# Autodesk Inventor assembly: Assembly1
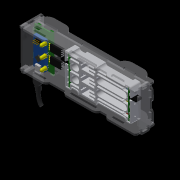
[picture p0: Inventor's stored thumbnail of the model, 180x180]
Saved by Autodesk Inventor 2016 (Build 200138000, 138)
## iProperties
Created: 2015-06-16
Part Number: Assembly1
Document SubType Name: Assembly
Designer: Openlab
Author: Openlab
## Documents named in this file (12)
- D:\Alexey\HS-Spectrophotometer\parts\Paris\Assembly.iam
- D:\Alexey\HS-Spectrophotometer\parts\Paris\Core_bottom.ipt
- D:\Alexey\HS-Spectrophotometer\parts\Paris\LED_board.ipt
- D:\Alexey\HS-Spectrophotometer\parts\Paris\Sensor_board.ipt
- D:\Alexey\HS-Spectrophotometer\parts\Paris\Core_top.ipt
- D:\Alexey\HS-Spectrophotometer\parts\Paris\Box_top.ipt
- D:\Alexey\HS-Spectrophotometer\parts\Paris\Box_bottom.ipt
- D:\Alexey\HS-Spectrophotometer\parts\Paris\Box_left_wall.ipt
- D:\Alexey\HS-Spectrophotometer\parts\Paris\Box_right_wall.ipt
- D:\Alexey\HS-Spectrophotometer\parts\Paris\Microcontroller_board_assumbly.iam
- D:\Alexey\HS-Spectrophotometer\parts\Paris\Box_back_wall.ipt
- D:\Alexey\HS-Spectrophotometer\parts\Paris\Box_front_wall.ipt
## Components (12 placed, 11 different names)
1. Core_bottom:1 — Mate:1, Mate:4, Mate:7, Mate:13, Mate:14, Mate:15, Mate:16, Mate:52, Mate:53, Mate:54, Mate:74
2. LED_board:1 — Mate:4, Mate:13, Mate:14
3. Sensor_board:1 — Mate:7, Mate:15, Mate:16
4. Core_top:1 — Mate:1, Mate:52, Mate:53, Mate:54, Mate:73, Mate:75
5. Box_top:1 — Mate:72, Mate:73, Mate:74, Mate:75, Mate:76, Mate:77, Mate:78, Mate:84, Mate:86, Mate:92
6. Box_bottom:1 — Mate:79, Mate:80, Mate:81
7. Box_left_wall:1 — Mate:83, Mate:84, Mate:85, Mate:91
8. Box_right_wall:1 — Mate:72
9. Microcontroller_board_assumbly:1 [sub-assembly] — Mate:89, Mate:90, Mate:91
10. Box_back_wall:1 — Mate:76, Mate:77, Mate:78, Mate:79, Mate:80, Mate:81, Mate:83, Mate:85, Mate:87, Mate:88
11. Box_front_wall:1 — Mate:92, Mate:93, Mate:94
12. Box_left_wall:2 — Mate:86, Mate:87, Mate:88, Mate:89, Mate:90, Mate:93, Mate:94
## Relationships (32: Mate 32)
- Mate:1: Core_bottom:1 ↔ Core_top:1
- Mate:4: Core_bottom:1 ↔ LED_board:1
- Mate:7: Core_bottom:1 ↔ Sensor_board:1
- Mate:13: Core_bottom:1 ↔ LED_board:1
- Mate:14: Core_bottom:1 ↔ LED_board:1
- Mate:15: Core_bottom:1 ↔ Sensor_board:1
- Mate:16: Core_bottom:1 ↔ Sensor_board:1
- Mate:52: Core_bottom:1 ↔ Core_top:1
- Mate:53: Core_bottom:1 ↔ Core_top:1
- Mate:54: Core_bottom:1 ↔ Core_top:1
- Mate:72: Box_top:1 ↔ Box_right_wall:1
- Mate:73: Core_top:1 ↔ Box_top:1
- Mate:74: Core_bottom:1 ↔ Box_top:1
- Mate:75: Core_top:1 ↔ Box_top:1
- Mate:76: Box_top:1 ↔ Box_back_wall:1
- Mate:77: Box_top:1 ↔ Box_back_wall:1
- Mate:78: Box_top:1 ↔ Box_back_wall:1
- Mate:79: Box_bottom:1 ↔ Box_back_wall:1
- Mate:80: Box_bottom:1 ↔ Box_back_wall:1
- Mate:81: Box_bottom:1 ↔ Box_back_wall:1
- Mate:83: Box_left_wall:1 ↔ Box_back_wall:1
- Mate:84: Box_top:1 ↔ Box_left_wall:1
- Mate:85: Box_left_wall:1 ↔ Box_back_wall:1
- Mate:86: Box_top:1 ↔ Box_left_wall:2
- Mate:87: Box_back_wall:1 ↔ Box_left_wall:2
- Mate:88: Box_back_wall:1 ↔ Box_left_wall:2
- Mate:89: Microcontroller_board_assumbly:1 ↔ Box_left_wall:2
- Mate:90: Microcontroller_board_assumbly:1 ↔ Box_left_wall:2
- Mate:91: Box_left_wall:1 ↔ Microcontroller_board_assumbly:1
- Mate:92: Box_top:1 ↔ Box_front_wall:1
- Mate:93: Box_front_wall:1 ↔ Box_left_wall:2
- Mate:94: Box_front_wall:1 ↔ Box_left_wall:2
